# Autodesk Inventor assembly: pulley 48 tooth + hub
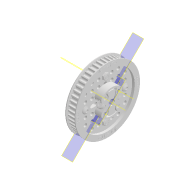
[picture p0: Inventor's stored thumbnail of the model, 180x180]
Saved by Autodesk Inventor 2020 (Build 240168000, 168)
## iProperties
Created: 2020-02-22
Part Number: pulley 48 tooth + hub
Document SubType Name: Assembly
Designer: ball
Author: ball
## Documents named in this file (3)
- C:\FTC\FTC8863CAD\2019 Robot\Mecanum Drive Train Metal\pulley 48 tooth + hub.iam
- C:\FTC\FTC8863CAD\GoBilda\3415 Parts\3415-0014-0048 Assembly.ipt
- C:\FTC\FTC8863CAD\GoBilda\1309 Parts\1309-0016-4008 assembly.ipt
## Components (2 placed, 2 different names)
1. 3415-0014-0048 Assembly:1 — Mate:1, Mate:2, Flush:1
2. 1309-0016-4008 assembly:1 — Mate:1, Mate:2, Flush:1
## Relationships (3: Mate 2, Flush 1)
- Mate:1: 3415-0014-0048 Assembly:1 ↔ 1309-0016-4008 assembly:1
- Mate:2: 3415-0014-0048 Assembly:1 ↔ 1309-0016-4008 assembly:1
- Flush:1: 3415-0014-0048 Assembly:1 ↔ 1309-0016-4008 assembly:1
